# Autodesk Inventor assembly: Test Prints
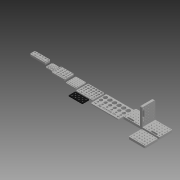
[picture p0: Inventor's stored thumbnail of the model, 180x180]
Saved by Autodesk Inventor 2022 (Build 260153000, 153)
## iProperties
Created: 2022-01-28
Part Number: Test Prints
Document SubType Name: Assembly
Designer: Cal
Author: Cal
## Documents named in this file (9)
- C:\Users\Cal\Desktop\Robotics\Design\Collaborative\Collaborative Parts Library\Tooling\Test Prints\Test Prints.iam
- C:\Users\Cal\Desktop\Robotics\Design\Collaborative\Collaborative Parts Library\Tooling\Test Prints\Bearing Test Print.ipt
- C:\Users\Cal\Desktop\Robotics\Design\Collaborative\Collaborative Parts Library\Tooling\Test Prints\Clearance Test Print.ipt
- C:\Users\Cal\Desktop\Robotics\Design\Collaborative\Collaborative Parts Library\Tooling\Test Prints\Drill Bushings Test Print.ipt
- C:\Users\Cal\Desktop\Robotics\Design\Collaborative\Collaborative Parts Library\Tooling\Test Prints\Hex Test Print.ipt
- C:\Users\Cal\Desktop\Robotics\Design\Collaborative\Collaborative Parts Library\Tooling\Test Prints\Hex Tolarance Guage.ipt
- C:\Users\Cal\Desktop\Robotics\Design\Collaborative\Collaborative Parts Library\Tooling\Test Prints\Nut Test Print.ipt
- C:\Users\Cal\Desktop\Robotics\Design\Collaborative\Collaborative Parts Library\Tooling\Test Prints\Tapped Test Print.ipt
- C:\Users\Cal\Desktop\Robotics\Design\Collaborative\Collaborative Parts Library\Tooling\Test Prints\Threaded Insert Test Print.ipt
## Components (9 placed, 8 different names)
1. Bearing Test Print:1 — Flush:1, Flush:9, Mate:18, Mate:19
2. Clearance Test Print:1 — Flush:1, Flush:2, Flush:9, Flush:10, Mate:22, Mate:23
3. Drill Bushings Test Print:1 — Flush:2, Flush:3, Flush:10, Flush:11, Mate:17, Mate:23
4. Hex Test Print:1 — Flush:3, Flush:4, Flush:11, Flush:12, Mate:1, Mate:16, Mate:19, Mate:20
5. Hex Tolarance Guage:1 — Flush:8, Mate:1, Mate:16
6. Nut Test Print:1 — Flush:4, Flush:5, Flush:8, Flush:12, Flush:13, Mate:21, Mate:22
7. Tapped Test Print:1 — Flush:5, Flush:6, Flush:13, Flush:15, Mate:20, Mate:21
8. Threaded Insert Test Print:1 — Flush:6, Flush:7, Mate:15, Flush:16
9. Threaded Insert Test Print:2 — Flush:7, Flush:15, Mate:15, Flush:16, Mate:18
## Relationships (25: Flush 15, Mate 10)
- Flush:1: Bearing Test Print:1 ↔ Clearance Test Print:1
- Flush:2: Clearance Test Print:1 ↔ Drill Bushings Test Print:1
- Flush:3: Drill Bushings Test Print:1 ↔ Hex Test Print:1
- Flush:4: Hex Test Print:1 ↔ Nut Test Print:1
- Flush:5: Nut Test Print:1 ↔ Tapped Test Print:1
- Flush:6: Tapped Test Print:1 ↔ Threaded Insert Test Print:1
- Flush:7: Threaded Insert Test Print:1 ↔ Threaded Insert Test Print:2
- Flush:8: Hex Tolarance Guage:1 ↔ Nut Test Print:1
- Flush:9: Bearing Test Print:1 ↔ Clearance Test Print:1
- Flush:10: Clearance Test Print:1 ↔ Drill Bushings Test Print:1
- Flush:11: Drill Bushings Test Print:1 ↔ Hex Test Print:1
- Flush:12: Hex Test Print:1 ↔ Nut Test Print:1
- Flush:13: Nut Test Print:1 ↔ Tapped Test Print:1
- Mate:15 (12.7 mm): Threaded Insert Test Print:1 ↔ Threaded Insert Test Print:2
- Flush:15: Tapped Test Print:1 ↔ Threaded Insert Test Print:2
- Mate:1 (12.7 mm): Hex Test Print:1 ↔ Hex Tolarance Guage:1
- Mate:16: Hex Test Print:1 ↔ Hex Tolarance Guage:1
- Flush:16: Threaded Insert Test Print:1 ↔ Threaded Insert Test Print:2
- Mate:17: Drill Bushings Test Print:1
- Mate:18 (12.7 mm): Bearing Test Print:1 ↔ Threaded Insert Test Print:2
- Mate:19 (12.7 mm): Bearing Test Print:1 ↔ Hex Test Print:1
- Mate:20 (12.7 mm): Hex Test Print:1 ↔ Tapped Test Print:1
- Mate:21 (12.7 mm): Nut Test Print:1 ↔ Tapped Test Print:1
- Mate:22 (12.7 mm): Clearance Test Print:1 ↔ Nut Test Print:1
- Mate:23 (12.7 mm): Clearance Test Print:1 ↔ Drill Bushings Test Print:1
